# Autodesk Inventor assembly: CIM for Ballshifter
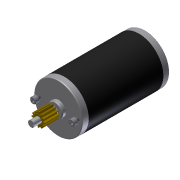
[picture p0: Inventor's stored thumbnail of the model, 180x180]
Saved by Autodesk Inventor 2013 (Build 170138000, 138)
## iProperties
Created: 2013-04-08
Part Number: CIM for Ballshifter
Document SubType Name: Assembly
Designer: Niemitalo_Dan
Author: Niemitalo_Dan
## Documents named in this file (4)
- \\lmss\students\Robotics\CAD Files\COTS Parts\Gearboxes\Components\VexPro Ballshifter Components\CIM for Ballshifter.iam
- \\lmss\students\Robotics\CAD Files\COTS Parts\Motors\CIM motor.ipt
- \\lmss\students\Robotics\CAD Files\COTS Parts\Gears - VexPro\Gear 20dp 10mm key 12T Vex.ipt
- \\lmss\students\Robotics\CAD Files\COTS Parts\Fasteners\10-32 SHCS x500.ipt
## Components (4 placed, 3 different names)
1. CIM motor:1 — Mate:1, Angle:1, Insert:1, Insert:2, Mate:2
2. Gear 20dp 10mm key 12T Vex:1 — Mate:1, Angle:1, Mate:2
3. 10-32 SHCS x500:1 — Insert:1
4. 10-32 SHCS x500:2 — Insert:2
## Relationships (5: Mate 2, Insert 2, Angle 1)
- Mate:1: CIM motor:1 ↔ Gear 20dp 10mm key 12T Vex:1
- Angle:1 (0 deg): CIM motor:1 ↔ Gear 20dp 10mm key 12T Vex:1
- Insert:1 (3.175 mm): CIM motor:1 ↔ 10-32 SHCS x500:1
- Insert:2 (3.175 mm): CIM motor:1 ↔ 10-32 SHCS x500:2
- Mate:2 (3.175 mm): CIM motor:1 ↔ Gear 20dp 10mm key 12T Vex:1
